# Autodesk Inventor assembly: fc18-054
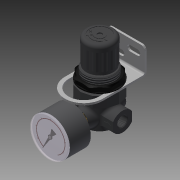
[picture p0: Inventor's stored thumbnail of the model, 180x180]
Saved by Autodesk Inventor 2018 (Build 220112000, 112)
## iProperties
Category: Pneumatics
Company: Autodesk Inc.
Created: 2017-11-24
Part Number: fc18-054
Document SubType Name: Assembly
Designer: Autodesk Inc.
Catalog Web Link: http://store.norgren.com/us/en/search.aspx?q=r07-100-rnea
Vendor: Norgren
Description: Main Regulator (assembled)
Author: Autodesk Inc.
Keywords: FIRST Choice
## Documents named in this file (5)
- F:\FIRST 2018\FIRST 2018 FirstChoice\fc18-054_MountKit.iam
- F:\FIRST 2018\FIRST 2018 FirstChoice\Parts\Pneumatics_Norgren_R07-100-RNEA.ipt
- F:\FIRST 2018\FIRST 2018 FirstChoice\Parts\Pneumatics_Norgren_18-025-003_Bracket.ipt
- F:\FIRST 2018\FIRST 2018 FirstChoice\Parts\Pneumatics_Norgren_18-025-003_Panel Nut.ipt
- F:\FIRST 2018\FIRST 2018 FirstChoice\Parts\Pneu_Norgren_18-013-212.iam
## Components (4 placed, 4 different names)
1. Pneumatics_Norgren_R07-100-RNEA:1 — Mate:1, Mate:2, Mate:3, Insert:1
2. Pneumatics_Norgren_18-025-003_Bracket:1 — Mate:1, Mate:2, Mate:4
3. Pneumatics_Norgren_18-025-003_Panel Nut:1 — Mate:3, Mate:4
4. Pneu_Norgren_18-013-212:1 [sub-assembly] — Insert:1
## Relationships (5: Mate 4, Insert 1)
- Mate:1: Pneumatics_Norgren_R07-100-RNEA:1 ↔ Pneumatics_Norgren_18-025-003_Bracket:1
- Mate:2: Pneumatics_Norgren_R07-100-RNEA:1 ↔ Pneumatics_Norgren_18-025-003_Bracket:1
- Mate:3: Pneumatics_Norgren_R07-100-RNEA:1 ↔ Pneumatics_Norgren_18-025-003_Panel Nut:1
- Mate:4: Pneumatics_Norgren_18-025-003_Bracket:1 ↔ Pneumatics_Norgren_18-025-003_Panel Nut:1
- Insert:1: Pneumatics_Norgren_R07-100-RNEA:1 ↔ Pneu_Norgren_18-013-212:1
